# Autodesk Inventor assembly: climber-assy
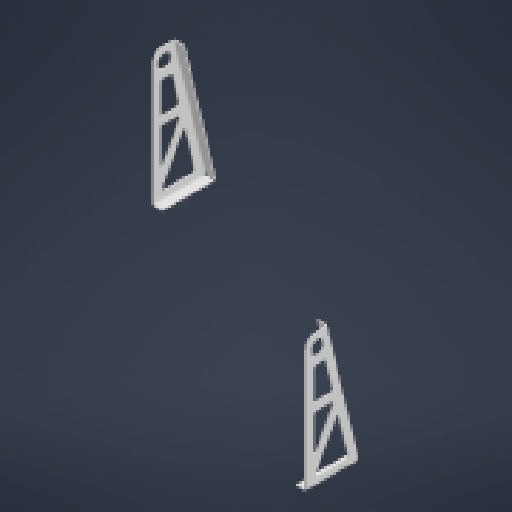
[picture p0: Inventor's stored thumbnail of the model, 512x512]
Saved by Autodesk Inventor 2025.1 (Build 291241020, 241B)
## iProperties
Category: _
Manager: _
ILogicPurgeVersion: 0.0.0.0
OnSaveVersion: 3.2.6.0
OnSaveAssembly: COREAutomationManager
Created: 2025-03-18
Part Number: climber-assy
Checked By: 00
Engr Approved By: _
User Status: Work In Process
Description: ASSY,STANDARD (mm)
Document SubType Name: Assembly
Mfg Approved By: Paul.Struhar
Designer: mathe
Mass: 1273.29 g
Surface Area: 4984.49 cm^2
Volume: 545.281 cm^3
Density: 2.3351 g/cm^3
CN_MASS: 0
CN_SERVICEABLE: _
FIRST_DESCRIPTION: _
SECOND_DESCRIPTION: _
THIRD_DESCRIPTION: _
CL_runCount: 0
ModelCat: Uncategorized
Subject: _
Author: mathe
Keywords: -
Revision Number: A
## Documents named in this file (5)
- D:\Documents\Inventor\2025-Poseidon-Mechanical\climber-assy.iam
- D:\Documents\Inventor\2025-Poseidon-Mechanical\Climber support.ipt
- D:\Documents\Inventor\2025-Poseidon-Mechanical\Climber support_MIR.ipt
- D:\Documents\Inventor\2025-Poseidon-Mechanical\climber-axle.ipt
- D:\Documents\Inventor\2025-Poseidon-Mechanical\grapplinghook.iam
## Components (4 placed, 4 different names)
1. Climber support:1 — Mate:1, Flush:1, Mate:2, Flush:2, Flush:3, Mate:3, Insert:1, Insert:2
2. Climber support_MIR:1 — Flush:2, Flush:3, Mate:3
3. climber-axle:1 — Insert:1
4. grapplinghook:1 [sub-assembly] — Insert:2
## Relationships (8: Mate 3, Flush 3, Insert 2)
- Mate:1: Climber support:1
- Flush:1: Climber support:1
- Mate:2: Climber support:1
- Flush:2: Climber support:1 ↔ Climber support_MIR:1
- Flush:3: Climber support:1 ↔ Climber support_MIR:1
- Mate:3 (325.12 mm): Climber support:1 ↔ Climber support_MIR:1
- Insert:1: Climber support:1 ↔ climber-axle:1
- Insert:2 (133.35 mm): Climber support:1 ↔ grapplinghook:1
